# Autodesk Inventor assembly: Engranaje-Planetario-Montaje
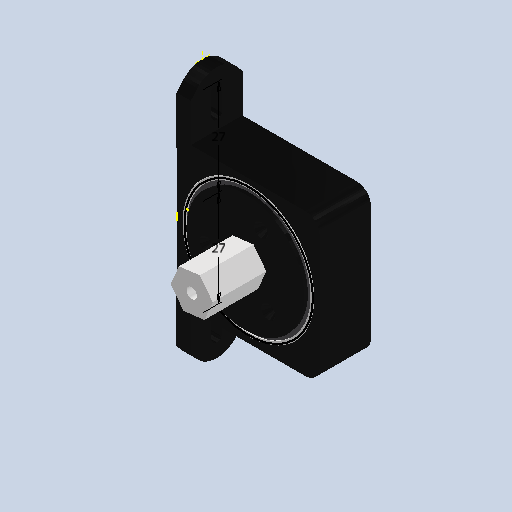
[picture p0: Inventor's stored thumbnail of the model, 512x512]
Saved by Autodesk Inventor 2024.2 (Build 282272000, 272)
## iProperties
Created: 2023-11-20
Part Number: Engranaje-Planetario-Montaje
Document SubType Name: Assembly
Designer: felip
Author: felip
## Documents named in this file (7)
- C:\Users\felip\Documentos\Robocupp-Mecanica\Gemelo Digital V2\Engranaje-Planetario-Montaje.iam
- C:\Users\felip\Documentos\Robocupp-Mecanica\Gemelo Digital V2\planetary_gearbox_rueda_exterior_ipt2.ipt
- C:\Users\felip\Documentos\Robocupp-Mecanica\Gemelo Digital V2\output_wheel_ipt2.ipt
- C:\Users\felip\Documentos\Robocupp-Mecanica\Gemelo Digital V2\input_wheel_ipt2.ipt
- C:\Users\felip\Documentos\Robocupp-Mecanica\Gemelo Digital V2\AST_Bearings_6706-2RS.ipt
- C:\Users\felip\Documentos\Robocupp-Mecanica\Gemelo Digital V2\ball bearing 6701 61701.ipt
- C:\Users\felip\Documentos\Robocupp-Mecanica\Gemelo Digital V2\Processed_SunGearV3.ipt
## Components (7 placed, 6 different names)
1. planetary_gearbox_rueda_exterior_ipt2:1 — Rotational:1, Rotational:2
2. output_wheel_ipt2:1 — Rotational:3
3. input_wheel_ipt2:1 — Rotational:4, Rotational:5
4. AST_Bearings_6706-2RS:1 — Rotational:2, Rotational:4
5. ball bearing 6701 61701:1 — Rigid:1, Rotational:5
6. Processed_SunGearV3:1 — Rigid:1
7. AST_Bearings_6706-2RS:2 — Rotational:1, Rotational:3
## Relationships (6: RevoluteJoint 5, WeldJoint 1)
- Rotational:1 [RevoluteJoint] (-4 mm): planetary_gearbox_rueda_exterior_ipt2:1 ↔ AST_Bearings_6706-2RS:2
- Rotational:2 [RevoluteJoint] (-4 mm): planetary_gearbox_rueda_exterior_ipt2:1 ↔ AST_Bearings_6706-2RS:1
- Rigid:1 [WeldJoint] (-10 mm): ball bearing 6701 61701:1 ↔ Processed_SunGearV3:1
- Rotational:3 [RevoluteJoint] (1 mm): output_wheel_ipt2:1 ↔ AST_Bearings_6706-2RS:2
- Rotational:4 [RevoluteJoint] (-1 mm): input_wheel_ipt2:1 ↔ AST_Bearings_6706-2RS:1
- Rotational:5 [RevoluteJoint] (-3.8 mm): input_wheel_ipt2:1 ↔ ball bearing 6701 61701:1
